# Autodesk Inventor assembly: TopMech
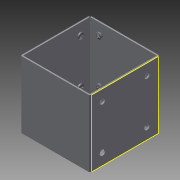
[picture p0: Inventor's stored thumbnail of the model, 180x180]
Saved by Autodesk Inventor 2013 (Build 170138000, 138)
## iProperties
Created: 2013-07-15
Part Number: TopMech
Document SubType Name: Assembly
Designer: root
Author: root
## Documents named in this file (5)
- I:\FRC_Projects\Cad\Inventor_Projects\Shooter-Cleaned\HopperAssembly\TopHopper\BoxwithSupport\BoxWIthSUpport.iam
- I:\FRC_Projects\Cad\Inventor_Projects\Shooter-Cleaned\HopperAssembly\TopHopper\BoxwithSupport\Box.ipt
- I:\FRC_Projects\Cad\Inventor_Projects\Shooter-Cleaned\HopperAssembly\TopHopper\BoxwithSupport\SideSupport.ipt
- I:\FRC_Projects\Cad\Inventor_Projects\Shooter-Cleaned\Libraries\ContentCenter\ANSI B18.6.3 - 5-44 UNF - 0.375(17).ipt
- I:\FRC_Projects\Cad\Inventor_Projects\Shooter-Cleaned\Libraries\ContentCenter\ANSI B18.6.3 - 5 - 44(2).ipt
## Components (11 placed, 4 different names)
1. Box:1 — Mate:1, Mate:2, Mate:3, Mate:4, Mate:5, Mate:6, Mate:7, Mate:9, Mate:10, Mate:13, Mate:14, Mate:15
2. SideSupport:1 — Mate:1, Mate:2, Mate:3, Mate:4, Mate:8, Mate:11, Mate:22, Mate:23
3. SideSupport:2 — Mate:5, Mate:6, Mate:7, Mate:12, Mate:20, Mate:21
4. Cross Recessed Binding Head Machine Screw - Type II - Inch No. 5 - 44 - 3/8:1 — Mate:8, Mate:9, Mate:16
5. Cross Recessed Binding Head Machine Screw - Type II - Inch No. 5 - 44 - 3/8:2 — Mate:11, Mate:13, Mate:17
6. Cross Recessed Binding Head Machine Screw - Type II - Inch No. 5 - 44 - 3/8:3 — Mate:12, Mate:14, Mate:18
7. Cross Recessed Binding Head Machine Screw - Type II - Inch No. 5 - 44 - 3/8:4 — Mate:10, Mate:15, Mate:19
8. Hex Machine Screw Nut - Inch 5 - 44:1 — Mate:16, Mate:22
9. Hex Machine Screw Nut - Inch 5 - 44:2 — Mate:17, Mate:23
10. Hex Machine Screw Nut - Inch 5 - 44:3 — Mate:18, Mate:21
11. Hex Machine Screw Nut - Inch 5 - 44:4 — Mate:19, Mate:20
## Relationships (23: Mate 23)
- Mate:1: Box:1 ↔ SideSupport:1
- Mate:2: Box:1 ↔ SideSupport:1
- Mate:3: Box:1 ↔ SideSupport:1
- Mate:4: Box:1 ↔ SideSupport:1
- Mate:5: Box:1 ↔ SideSupport:2
- Mate:6: Box:1 ↔ SideSupport:2
- Mate:7: Box:1 ↔ SideSupport:2
- Mate:8: SideSupport:1 ↔ Cross Recessed Binding Head Machine Screw - Type II - Inch No. 5 - 44 - 3/8:1
- Mate:9: Box:1 ↔ Cross Recessed Binding Head Machine Screw - Type II - Inch No. 5 - 44 - 3/8:1
- Mate:10: Box:1 ↔ Cross Recessed Binding Head Machine Screw - Type II - Inch No. 5 - 44 - 3/8:4
- Mate:11: SideSupport:1 ↔ Cross Recessed Binding Head Machine Screw - Type II - Inch No. 5 - 44 - 3/8:2
- Mate:12: SideSupport:2 ↔ Cross Recessed Binding Head Machine Screw - Type II - Inch No. 5 - 44 - 3/8:3
- Mate:13: Box:1 ↔ Cross Recessed Binding Head Machine Screw - Type II - Inch No. 5 - 44 - 3/8:2
- Mate:14: Box:1 ↔ Cross Recessed Binding Head Machine Screw - Type II - Inch No. 5 - 44 - 3/8:3
- Mate:15: Box:1 ↔ Cross Recessed Binding Head Machine Screw - Type II - Inch No. 5 - 44 - 3/8:4
- Mate:16: Cross Recessed Binding Head Machine Screw - Type II - Inch No. 5 - 44 - 3/8:1 ↔ Hex Machine Screw Nut - Inch 5 - 44:1
- Mate:17: Cross Recessed Binding Head Machine Screw - Type II - Inch No. 5 - 44 - 3/8:2 ↔ Hex Machine Screw Nut - Inch 5 - 44:2
- Mate:18: Cross Recessed Binding Head Machine Screw - Type II - Inch No. 5 - 44 - 3/8:3 ↔ Hex Machine Screw Nut - Inch 5 - 44:3
- Mate:19: Cross Recessed Binding Head Machine Screw - Type II - Inch No. 5 - 44 - 3/8:4 ↔ Hex Machine Screw Nut - Inch 5 - 44:4
- Mate:20: SideSupport:2 ↔ Hex Machine Screw Nut - Inch 5 - 44:4
- Mate:21: SideSupport:2 ↔ Hex Machine Screw Nut - Inch 5 - 44:3
- Mate:22: SideSupport:1 ↔ Hex Machine Screw Nut - Inch 5 - 44:1
- Mate:23: SideSupport:1 ↔ Hex Machine Screw Nut - Inch 5 - 44:2
